# Autodesk Inventor assembly: 2AM-17-A-6200 - claw arm
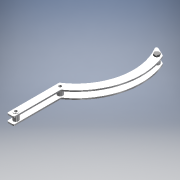
[picture p0: Inventor's stored thumbnail of the model, 180x180]
Saved by Autodesk Inventor 2017 (Build 210142000, 142)
## iProperties
Created: 2017-12-27
Part Number: 2AM-17-A-6200 - claw arm
Document SubType Name: Assembly
Designer: Micah
Mass: 120.47 g
Surface Area: 321.031 cm^2
Volume: 41.585 cm^3
Density: 2.89695 g/cm^3
Author: Micah
## Documents named in this file (6)
- C:\Users\Micah\Desktop\inventor\CADathon-2017\2AM-17-A-0200 - Smokestack Elevator\2AM-17-A-6200 - claw arm.iam
- C:\Users\Micah\Desktop\inventor\CADathon-2017\2AM-17-A-0200 - Smokestack Elevator\2AM-17-P-5201 - claw arm.ipt
- C:\Users\Micah\Desktop\inventor\CADathon-2017\2AM-17-A-0200 - Smokestack Elevator\2AM-17-P-5202 - arm supports.ipt
- C:\Users\Micah\Documents\Inventor\Content Center Files\R2017\en-US\AS 2465(2)\AS 2465 - 1_4 x 1  UNC.ipt
- C:\Users\Micah\Documents\Inventor\Content Center Files\R2017\en-US\AS 2465(3)\AS 2465 - 1_4  UNC(2).ipt
- C:\Users\Micah\Desktop\inventor\CADathon-2017\2AM-17-A-0200 - Smokestack Elevator\2AM-17-P-5206 - spacer 035.ipt
## Components (9 placed, 5 different names)
1. 2AM-17-P-5201 - claw arm:1 — Mate:4, Insert:3, Mate:5
2. 2AM-17-P-5201 - claw arm:2 — Mate:1, Mate:2, Mate:3, Insert:6, Mate:6
3. 2AM-17-P-5202 - arm supports:1 — Mate:1, Mate:4
4. 2AM-17-P-5202 - arm supports:2 — Mate:2
5. 2AM-17-P-5202 - arm supports:3 — Mate:3
6. AS 2465 - Inch 1/4 x 1  UNC:3 — Insert:3
7. AS 2465 (Unified hexagon bolts, screws and nuts (UNC and UNF threads) - Inch 1/4  UNC:3 — Insert:6
8. 2AM-17-P-5206 - spacer 035:1 — Mate:5
9. 2AM-17-P-5206 - spacer 035:2 — Mate:6
## Relationships (8: Mate 6, Insert 2)
- Mate:1: 2AM-17-P-5201 - claw arm:2 ↔ 2AM-17-P-5202 - arm supports:1
- Mate:2: 2AM-17-P-5201 - claw arm:2 ↔ 2AM-17-P-5202 - arm supports:2
- Mate:3: 2AM-17-P-5201 - claw arm:2 ↔ 2AM-17-P-5202 - arm supports:3
- Mate:4: 2AM-17-P-5201 - claw arm:1 ↔ 2AM-17-P-5202 - arm supports:1
- Insert:3: 2AM-17-P-5201 - claw arm:1 ↔ AS 2465 - Inch 1/4 x 1  UNC:3
- Insert:6: 2AM-17-P-5201 - claw arm:2 ↔ AS 2465 (Unified hexagon bolts, screws and nuts (UNC and UNF threads) - Inch 1/4  UNC:3
- Mate:5: 2AM-17-P-5201 - claw arm:1 ↔ 2AM-17-P-5206 - spacer 035:1
- Mate:6: 2AM-17-P-5201 - claw arm:2 ↔ 2AM-17-P-5206 - spacer 035:2
